# Autodesk Inventor assembly: Rear Piston_MIR
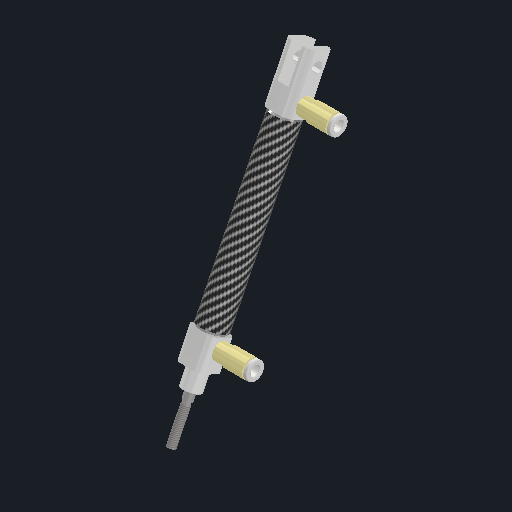
[picture p0: Inventor's stored thumbnail of the model, 512x512]
Saved by Autodesk Inventor 2025 (Build 290162000, 162)
## iProperties
Created: 2025-01-04
Part Number: Rear Piston_MIR
Document SubType Name: Assembly
Designer: Juan
Author: Juan
## Documents named in this file (4)
- C:\Users\Juan\Documents\GitHub\ATUM-VRC-High-Stakes-CAD\Robot\Subassemblies\Rear Piston_MIR.iam
- C:\Users\Juan\Documents\GitHub\ATUM-VRC-High-Stakes-CAD\VEX-CAD-Inventor\Motion\Pneumatics\Reference Parts\Pistons\Double Acting Piston Body_MIR.ipt
- C:\Users\Juan\Documents\GitHub\ATUM-VRC-High-Stakes-CAD\VEX-CAD-Inventor\Motion\Pneumatics\Reference Parts\Pistons\Double Acting Piston Rod_MIR.ipt
- C:\Users\Juan\Documents\GitHub\ATUM-VRC-High-Stakes-CAD\VEX-CAD-Inventor\Motion\Pneumatics\Legacy - SMC Pneumatics\Fitting for Cylinders_MIR.ipt
## Components (4 placed, 3 different names)
1. Double Acting Piston Body_MIR:1 — Mate:1, Mate:4, Mate:3, Mate:5, Mate:2
2. Double Acting Piston Rod_MIR:1 — Mate:1
3. Fitting for Cylinders_MIR:1 — Mate:4, Mate:3
4. Fitting for Cylinders_MIR:2 — Mate:5, Mate:2
## Relationships (5: Mate 5)
- Mate:1: Double Acting Piston Body_MIR:1 ↔ Double Acting Piston Rod_MIR:1
- Mate:4: Double Acting Piston Body_MIR:1 ↔ Fitting for Cylinders_MIR:1
- Mate:3: Double Acting Piston Body_MIR:1 ↔ Fitting for Cylinders_MIR:1
- Mate:5: Double Acting Piston Body_MIR:1 ↔ Fitting for Cylinders_MIR:2
- Mate:2: Double Acting Piston Body_MIR:1 ↔ Fitting for Cylinders_MIR:2
